# Autodesk Inventor assembly: INNER TORSO
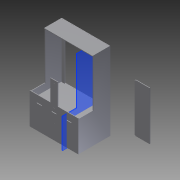
[picture p0: Inventor's stored thumbnail of the model, 180x180]
Saved by Autodesk Inventor 2011 (Build 150239000, 239)
## iProperties
Created: 2011-09-03
Part Number: INNER TORSO
Document SubType Name: Assembly
Designer: Matthew
Author: Matthew
## Documents named in this file (7)
- C:\Users\Matthew\Documents\matthew_autocad\prlite\inner torso\INNER TORSO.iam
- C:\Users\Matthew\Documents\matthew_autocad\prlite\inner torso\it back.ipt
- C:\Users\Matthew\Documents\matthew_autocad\prlite\inner torso\it side.ipt
- C:\Users\Matthew\Documents\matthew_autocad\prlite\inner torso\it front.ipt
- C:\Users\Matthew\Documents\matthew_autocad\prlite\inner torso\it top.ipt
- C:\Users\Matthew\Documents\matthew_autocad\prlite\inner torso\it bottom.ipt
- C:\Users\Matthew\Documents\matthew_autocad\prlite\inner torso\it shelf.ipt
## Components (7 placed, 6 different names)
1. it back:1 — Flush:9, Flush:12, Flush:13, Mate:4, Flush:14, Mate:13, Mate:14, Flush:22, Mate:17
2. it side:1 — Flush:5, Mate:7, Flush:18, Flush:19, Mate:13, Mate:18, Mate:19
3. it front:1 — Flush:5, Mate:7, Mate:11, Flush:17, Flush:19, Flush:23
4. it top:1 — Flush:9, Mate:17, Mate:19
5. it bottom:1 — Flush:12, Mate:11, Flush:17, Flush:18, Mate:15, Mate:18
6. it shelf:1 — Flush:13, Mate:4, Flush:14
7. it side:2 — Mate:14, Flush:22, Flush:23, Mate:15
## Relationships (19: Flush 10, Mate 9)
- Flush:5: it side:1 ↔ it front:1
- Flush:9: it back:1 ↔ it top:1
- Flush:12: it back:1 ↔ it bottom:1
- Flush:13: it back:1 ↔ it shelf:1
- Mate:4: it back:1 ↔ it shelf:1
- Flush:14: it back:1 ↔ it shelf:1
- Mate:7: it side:1 ↔ it front:1
- Mate:11: it front:1 ↔ it bottom:1
- Flush:17: it front:1 ↔ it bottom:1
- Flush:18: it side:1 ↔ it bottom:1
- Flush:19: it side:1 ↔ it front:1
- Mate:13: it back:1 ↔ it side:1
- Mate:14: it back:1 ↔ it side:2
- Flush:22: it back:1 ↔ it side:2
- Flush:23: it front:1 ↔ it side:2
- Mate:15: it bottom:1 ↔ it side:2
- Mate:17: it back:1 ↔ it top:1
- Mate:18: it side:1 ↔ it bottom:1
- Mate:19: it side:1 ↔ it top:1
